# Autodesk Inventor assembly: !Drivebay Right.I am
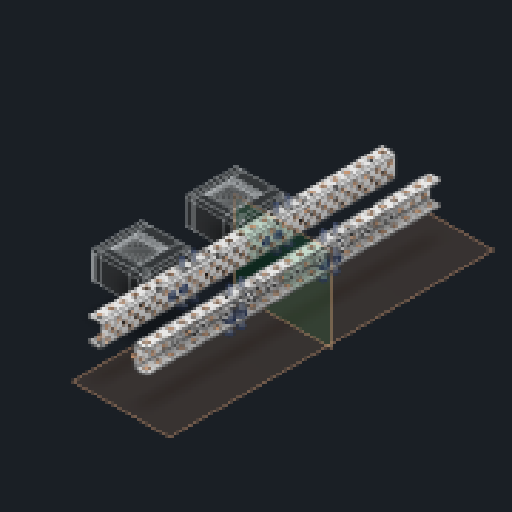
[picture p0: Inventor's stored thumbnail of the model, 512x512]
Saved by Autodesk Inventor 2025.1 (Build 291241000, 241)
## iProperties
Created: 2024-11-28
Part Number: !Drivebay Right.I am
Document SubType Name: Assembly
Designer: avere
Author: avere
## Documents named in this file (3)
- C:\Users\avere\VEX\High Stakes\CAD\Codie\Chassis\Drivebay Right\!Drivebay Right.I am.iam
- C:\Users\avere\VEX\High Stakes\CAD\Codie\Chassis\Drivebay Right\Outer.iam
- C:\Users\avere\VEX\High Stakes\CAD\Codie\Chassis\Drivebay Right\Inner.iam
## Components (2 placed, 2 different names)
1. Outer:1 [sub-assembly] — Flush:1, Mate:2, Mate:1
2. Inner:1 [sub-assembly] — Flush:3, Mate:3, Flush:2
## Relationships (6: Mate 4, Flush 2)
- Flush:1 [Mate] (-158.75 mm): Outer:1
- Mate:2 (41.275 mm): Outer:1
- Mate:1 (17.4625 mm): Outer:1
- Flush:3 (17.4625 mm): Inner:1
- Mate:3 (41.275 mm): Inner:1
- Flush:2 (-158.75 mm): Inner:1
